# Autodesk Inventor assembly: Montagem uwu
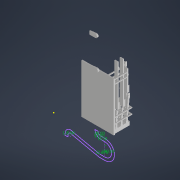
[picture p0: Inventor's stored thumbnail of the model, 180x180]
Saved by Autodesk Inventor 2022 (Build 260153000, 153)
## iProperties
Created: 2023-05-12
Part Number: Montagem uwu
Document SubType Name: Assembly
Designer: jpjoa
Author: jpjoa
## Documents named in this file (15)
- G:\My Drive\Faculdade\Trabalhos\Desenho e Print 3D\Marbles project\Montagem uwu.iam
- G:\My Drive\Faculdade\Trabalhos\Desenho e Print 3D\Marbles project\Agrupar bolinhas novamente.ipt
- G:\My Drive\Faculdade\Trabalhos\Desenho e Print 3D\Marbles project\Base.ipt
- G:\My Drive\Faculdade\Trabalhos\Desenho e Print 3D\Marbles project\Box de reinício.ipt
- G:\My Drive\Faculdade\Trabalhos\Desenho e Print 3D\Marbles project\Conector superior para giro.ipt
- G:\My Drive\Faculdade\Trabalhos\Desenho e Print 3D\Marbles project\Libera todas.ipt
- G:\My Drive\Faculdade\Trabalhos\Desenho e Print 3D\Marbles project\Pega uma e libera superior.ipt
- G:\My Drive\Faculdade\Trabalhos\Desenho e Print 3D\Marbles project\Pega uma e libera.ipt
- G:\My Drive\Faculdade\Trabalhos\Desenho e Print 3D\Marbles project\Receptor pequeno.ipt
- G:\My Drive\Faculdade\Trabalhos\Desenho e Print 3D\Marbles project\Receptor.ipt
- G:\My Drive\Faculdade\Trabalhos\Desenho e Print 3D\Marbles project\Sustentação Trilhos fixos.ipt
- G:\My Drive\Faculdade\Trabalhos\Desenho e Print 3D\Marbles project\Trilho 5 minutos.ipt
- G:\My Drive\Faculdade\Trabalhos\Desenho e Print 3D\Marbles project\Trilho 60 minutos  - 12 horas.ipt
- G:\My Drive\Faculdade\Trabalhos\Desenho e Print 3D\Marbles project\Troca de sentido.ipt
- G:\My Drive\Faculdade\Trabalhos\Desenho e Print 3D\Marbles project\Sustentação Trilhos.ipt
## Components (18 placed, 14 different names)
1. Agrupar bolinhas novamente:1
2. Base:1 — Coincidente:1, Alinhado:4, Coincidente:3, Coincidente:4, Coincidente:5, Ângulo:1, Coincidente:6, Alinhado:14, Ângulo:2, Ângulo:3, Ângulo:4, Coincidente:8, Alinhado:15
3. Box de reinício:1 — Coincidente:1, Inserir:1, Inserir:3, Alinhado:1, Alinhado:2, Alinhado:3, Alinhado:4, Inserir:12, Coincidente:7
4. Libera todas:1 — Inserir:3, Alinhado:3
5. Pega uma e libera superior:1 — Inserir:1, Alinhado:1, Alinhado:11, Alinhado:13
6. Pega uma e libera:1 — Alinhado:2, Inserir:12
7. Receptor pequeno:1
8. Receptor:1 — Inserir:5, Alinhado:7, Alinhado:9, Alinhado:10
9. Sustentação Trilhos fixos:1 — Coincidente:6, Coincidente:7, Alinhado:14
10. Trilho 5 minutos:1 — Inserir:4, Alinhado:6, Ângulo:2
11. Trilho 60 minutos  - 12 horas:1 — Inserir:5, Alinhado:7, Ângulo:3
12. Receptor:2 — Inserir:6, Alinhado:8, Alinhado:10
13. Receptor:3 — Inserir:4, Alinhado:6, Alinhado:9, Alinhado:11
14. Trilho 60 minutos  - 12 horas:2 — Inserir:6, Alinhado:8, Ângulo:4
15. Receptor pequeno:2
16. Conector superior para giro:1 — Inserir:11, Alinhado:12
17. Troca de sentido:1 — Inserir:11, Alinhado:12, Ângulo:1, Alinhado:13
18. Sustentação Trilhos:1 — Coincidente:8, Alinhado:15
## Relationships (32: Flush 14, Mate 7, Insert 7, Angle 4)
- Coincidente:1 [Mate]: Base:1 ↔ Box de reinício:1
- Inserir:1: Box de reinício:1 ↔ Pega uma e libera superior:1
- Inserir:3: Box de reinício:1 ↔ Libera todas:1
- Alinhado:1 [Flush]: Box de reinício:1 ↔ Pega uma e libera superior:1
- Alinhado:2 [Flush]: Box de reinício:1 ↔ Pega uma e libera:1
- Alinhado:3 [Flush]: Box de reinício:1 ↔ Libera todas:1
- Alinhado:4 [Flush]: Base:1 ↔ Box de reinício:1
- Inserir:4: Trilho 5 minutos:1 ↔ Receptor:3
- Alinhado:6 [Flush]: Trilho 5 minutos:1 ↔ Receptor:3
- Inserir:5: Receptor:1 ↔ Trilho 60 minutos  - 12 horas:1
- Alinhado:7 [Flush]: Receptor:1 ↔ Trilho 60 minutos  - 12 horas:1
- Inserir:6: Receptor:2 ↔ Trilho 60 minutos  - 12 horas:2
- Alinhado:8 [Flush]: Receptor:2 ↔ Trilho 60 minutos  - 12 horas:2
- Alinhado:9 [Flush]: Receptor:1 ↔ Receptor:3
- Alinhado:10 [Flush]: Receptor:1 ↔ Receptor:2
- Alinhado:11 [Flush]: Pega uma e libera superior:1 ↔ Receptor:3
- Coincidente:3 [Mate]: Base:1
- Coincidente:4 [Mate]: Base:1
- Coincidente:5 [Mate]: Base:1
- Inserir:11: Conector superior para giro:1 ↔ Troca de sentido:1
- Alinhado:12 [Flush]: Conector superior para giro:1 ↔ Troca de sentido:1
- Ângulo:1 [Angle] (180 deg): Base:1 ↔ Troca de sentido:1
- Alinhado:13 [Flush]: Pega uma e libera superior:1 ↔ Troca de sentido:1
- Inserir:12: Box de reinício:1 ↔ Pega uma e libera:1
- Coincidente:6 [Mate]: Base:1 ↔ Sustentação Trilhos fixos:1
- Coincidente:7 [Mate]: Box de reinício:1 ↔ Sustentação Trilhos fixos:1
- Alinhado:14 [Flush]: Base:1 ↔ Sustentação Trilhos fixos:1
- Ângulo:2 [Angle] (0 deg): Base:1 ↔ Trilho 5 minutos:1
- Ângulo:3 [Angle] (0 deg): Base:1 ↔ Trilho 60 minutos  - 12 horas:1
- Ângulo:4 [Angle] (0 deg): Base:1 ↔ Trilho 60 minutos  - 12 horas:2
- Coincidente:8 [Mate]: Base:1 ↔ Sustentação Trilhos:1
- Alinhado:15 [Flush]: Base:1 ↔ Sustentação Trilhos:1
